# Autodesk Inventor assembly: hand
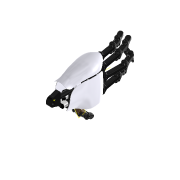
[picture p0: Inventor's stored thumbnail of the model, 180x180]
Saved by Autodesk Inventor 2020.2 (Build 242310000, 310)
## iProperties
Created: 2020-04-08
Part Number: hand
Document SubType Name: Assembly
Designer: Bardo91
thread_hole: 2.500 mm
Author: Bardo91
## Documents named in this file (23)
- D:\programming\bioarm\hardware\1. hand\elric20-1A.iam
- D:\programming\bioarm\hardware\1. hand\pinky_f1.ipt
- D:\programming\bioarm\hardware\1. hand\pinky_f2.ipt
- D:\programming\bioarm\hardware\1. hand\pinky_f3.ipt
- D:\programming\bioarm\hardware\1. hand\base_hand.ipt
- D:\programming\bioarm\hardware\1. hand\motor_dc_6v_30rpm.ipt
- D:\programming\bioarm\hardware\1. hand\finger_thread_lock.ipt
- D:\programming\bioarm\hardware\1. hand\finger_pulley.ipt
- D:\programming\bioarm\hardware\1. hand\ring_f2.ipt
- D:\programming\bioarm\hardware\1. hand\ring_f3.ipt
- D:\programming\bioarm\hardware\1. hand\ring_f1.ipt
- D:\programming\bioarm\hardware\1. hand\middle_f1.ipt
- D:\programming\bioarm\hardware\1. hand\middle_f2.ipt
- D:\programming\bioarm\hardware\1. hand\middle_f3.ipt
- D:\programming\bioarm\hardware\1. hand\index_f1.ipt
- D:\programming\bioarm\hardware\1. hand\index_f2.ipt
- D:\programming\bioarm\hardware\1. hand\index_f3.ipt
- D:\programming\bioarm\hardware\1. hand\thumb_f2.ipt
- D:\programming\bioarm\hardware\1. hand\thumb_f3.ipt
- D:\programming\bioarm\hardware\1. hand\thumb_f1.ipt
- D:\programming\bioarm\hardware\1. hand\cases\hand_case_1.ipt
- D:\programming\bioarm\hardware\1. hand\cases\hand_case_2.ipt
- D:\programming\bioarm\hardware\1. hand\cases\hand_case_3.ipt
## Components (31 placed, 22 different names)
1. base_hand:1 — Flush:9, Mate:12, Mate:32, Mate:33, Mate:36, Mate:37, Mate:40, Mate:41, Mate:48, Mate:49, Mate:50, Mate:51, Mate:52, Mate:53, Mate:54, Mate:55, Mate:56, Mate:57, Mate:58, Mate:59, Mate:64, Mate:65, Mate:69, Mate:70, Mate:71, Mate:72, Mate:73
2. hand_case_1:1 — Mate:73
3. hand_case_2:1
4. hand_case_3:1
5. motor_dc_6v_30rpm:1 — Mate:28, Mate:29, Mate:48, Mate:56, Mate:58
6. finger_thread_lock:1 — Mate:25, Mate:26
7. finger_pulley:1 — Mate:28, Mate:29
8. pinky_f1:1 — Mate:1, Flush:1, Flush:9, Mate:12
9. pinky_f2:1 — Mate:1, Flush:1, Flush:2, Mate:2
10. pinky_f3:1 — Flush:2, Mate:2, Mate:25, Mate:26
11. finger_pulley:4 — Mate:44, Mate:45
12. motor_dc_6v_30rpm:2 — Mate:44, Mate:45, Mate:49, Mate:55, Mate:57
13. ring_f2:1 — Mate:30, Mate:31, Flush:10, Flush:11
14. ring_f3:1 — Mate:30, Flush:10
15. ring_f1:1 — Mate:31, Flush:11, Mate:32, Mate:33
16. motor_dc_6v_30rpm:4 — Mate:42, Mate:47, Mate:50, Mate:54, Mate:59
17. finger_pulley:3 — Mate:43, Mate:46
18. middle_f1:1 — Mate:35, Mate:36, Mate:37, Flush:12
19. middle_f2:1 — Mate:34, Mate:35, Flush:12, Flush:13
20. middle_f3:1 — Mate:34, Flush:13
21. motor_dc_6v_30rpm:3 — Mate:43, Mate:46, Mate:51, Mate:52, Mate:53
22. finger_pulley:2 — Mate:42, Mate:47
23. index_f1:1 — Mate:39, Mate:40, Flush:15, Mate:41
24. index_f2:1 — Mate:38, Mate:39, Flush:14, Flush:15
25. index_f3:1 — Mate:38, Flush:14
26. motor_dc_6v_30rpm:5 — Mate:62, Mate:63, Mate:64, Mate:65, Mate:69
27. motor_dc_6v_30rpm:6 — Mate:67, Mate:68, Mate:70, Mate:71, Mate:72
28. finger_pulley:5 — Mate:67, Mate:68
29. thumb_f1:1 — Mate:61, Flush:17, Mate:62, Mate:63
30. thumb_f2:1 — Mate:60, Mate:61, Flush:16, Flush:17
31. thumb_f3:1 — Mate:60, Flush:16
## Relationships (61: Mate 50, Flush 11)
- Mate:1: pinky_f1:1 ↔ pinky_f2:1
- Flush:1: pinky_f1:1 ↔ pinky_f2:1
- Flush:2: pinky_f2:1 ↔ pinky_f3:1
- Mate:2: pinky_f2:1 ↔ pinky_f3:1
- Flush:9: base_hand:1 ↔ pinky_f1:1
- Mate:12: base_hand:1 ↔ pinky_f1:1
- Mate:25: finger_thread_lock:1 ↔ pinky_f3:1
- Mate:26 (0.25 mm): finger_thread_lock:1 ↔ pinky_f3:1
- Mate:28 (0.5 mm): motor_dc_6v_30rpm:1 ↔ finger_pulley:1
- Mate:29: motor_dc_6v_30rpm:1 ↔ finger_pulley:1
- Mate:30: ring_f2:1 ↔ ring_f3:1
- Mate:31: ring_f2:1 ↔ ring_f1:1
- Flush:10: ring_f2:1 ↔ ring_f3:1
- Flush:11: ring_f2:1 ↔ ring_f1:1
- Mate:32: base_hand:1 ↔ ring_f1:1
- Mate:33: base_hand:1 ↔ ring_f1:1
- Mate:34: middle_f2:1 ↔ middle_f3:1
- Mate:35: middle_f1:1 ↔ middle_f2:1
- Mate:36: base_hand:1 ↔ middle_f1:1
- Mate:37: base_hand:1 ↔ middle_f1:1
- Flush:12: middle_f1:1 ↔ middle_f2:1
- Flush:13: middle_f2:1 ↔ middle_f3:1
- Mate:38: index_f2:1 ↔ index_f3:1
- Mate:39: index_f1:1 ↔ index_f2:1
- Mate:40: base_hand:1 ↔ index_f1:1
- Flush:14: index_f2:1 ↔ index_f3:1
- Flush:15: index_f1:1 ↔ index_f2:1
- Mate:41: base_hand:1 ↔ index_f1:1
- Mate:42: motor_dc_6v_30rpm:4 ↔ finger_pulley:2
- Mate:43: finger_pulley:3 ↔ motor_dc_6v_30rpm:3
- Mate:44: finger_pulley:4 ↔ motor_dc_6v_30rpm:2
- Mate:45 (0.5 mm): finger_pulley:4 ↔ motor_dc_6v_30rpm:2
- Mate:46 (0.5 mm): finger_pulley:3 ↔ motor_dc_6v_30rpm:3
- Mate:47 (0.5 mm): motor_dc_6v_30rpm:4 ↔ finger_pulley:2
- Mate:48: base_hand:1 ↔ motor_dc_6v_30rpm:1
- Mate:49: base_hand:1 ↔ motor_dc_6v_30rpm:2
- Mate:50: base_hand:1 ↔ motor_dc_6v_30rpm:4
- Mate:51: base_hand:1 ↔ motor_dc_6v_30rpm:3
- Mate:52: base_hand:1 ↔ motor_dc_6v_30rpm:3
- Mate:53: base_hand:1 ↔ motor_dc_6v_30rpm:3
- Mate:54: base_hand:1 ↔ motor_dc_6v_30rpm:4
- Mate:55: base_hand:1 ↔ motor_dc_6v_30rpm:2
- Mate:56: base_hand:1 ↔ motor_dc_6v_30rpm:1
- Mate:57: base_hand:1 ↔ motor_dc_6v_30rpm:2
- Mate:58: base_hand:1 ↔ motor_dc_6v_30rpm:1
- Mate:59: base_hand:1 ↔ motor_dc_6v_30rpm:4
- Mate:60: thumb_f2:1 ↔ thumb_f3:1
- Mate:61: thumb_f1:1 ↔ thumb_f2:1
- Flush:16: thumb_f2:1 ↔ thumb_f3:1
- Flush:17: thumb_f1:1 ↔ thumb_f2:1
- Mate:62: motor_dc_6v_30rpm:5 ↔ thumb_f1:1
- Mate:63 (1 mm): motor_dc_6v_30rpm:5 ↔ thumb_f1:1
- Mate:64: base_hand:1 ↔ motor_dc_6v_30rpm:5
- Mate:65: base_hand:1 ↔ motor_dc_6v_30rpm:5
- Mate:67: motor_dc_6v_30rpm:6 ↔ finger_pulley:5
- Mate:68 (1 mm): motor_dc_6v_30rpm:6 ↔ finger_pulley:5
- Mate:69: base_hand:1 ↔ motor_dc_6v_30rpm:5
- Mate:70: base_hand:1 ↔ motor_dc_6v_30rpm:6
- Mate:71: base_hand:1 ↔ motor_dc_6v_30rpm:6
- Mate:72: base_hand:1 ↔ motor_dc_6v_30rpm:6
- Mate:73: base_hand:1 ↔ hand_case_1:1
## Named parameters: thread_hole = 2.5 mm
